# Autodesk Inventor assembly: prototype3
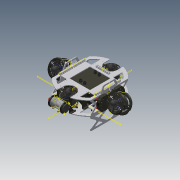
[picture p0: Inventor's stored thumbnail of the model, 180x180]
Saved by Autodesk Inventor 2018 (Build 220112000, 112)
## iProperties
Created: 2020-01-08
Part Number: prototype3
Document SubType Name: Assembly
Designer: anirudh
Author: anirudh
## Documents named in this file (33)
- D:\Silicon Sharks\2019-2020\prototype3\prototype3.iam
- D:\Silicon Sharks\2019-2020\prototype3\bottomPlate.ipt
- D:\Silicon Sharks\2019-2020\ElectronicsHousing\Prototype2\ElectricalHousing2.iam
- D:\Silicon Sharks\2019-2020\prototype3\servo.ipt
- D:\Silicon Sharks\2019-2020\prototype3\servoBracket.ipt
- D:\Silicon Sharks\2019-2020\prototype3\REV-41-1363.ipt
- D:\Silicon Sharks\2019-2020\prototype3\T200-THRUSTER.ipt
- D:\Silicon Sharks\2019-2020\prototype3\sidePlate.ipt
- D:\Silicon Sharks\2019-2020\prototype3\thrusterGimbalMount.ipt
- D:\Silicon Sharks\2019-2020\prototype3\thrusterMount.ipt
- D:\Silicon Sharks\2019-2020\prototype3\gimbalShroud.ipt
- D:\Silicon Sharks\2019-2020\prototype3\thrusterGuards.ipt
- D:\Silicon Sharks\2019-2020\prototype3\thrusterGuard2.ipt
- D:\Silicon Sharks\2019-2020\prototype3\verticalThrusterMount.ipt
- D:\Silicon Sharks\2019-2020\prototype3\topPlate.ipt
- D:\Silicon Sharks\2019-2020\CameraEnclosure\CameraEnclosure1.iam
- D:\Silicon Sharks\2019-2020\prototype3\cameraMount1.ipt
- D:\Silicon Sharks\2019-2020\prototype3\cameraMount2.ipt
- D:\Silicon Sharks\2019-2020\prototype3\cameraMount3.ipt
- D:\Silicon Sharks\2019-2020\prototype3\7inREV.ipt
- D:\Silicon Sharks\2019-2020\prototype3\4inREV.ipt
- D:\Silicon Sharks\2019-2020\prototype3\standoff.ipt
- D:\Silicon Sharks\2019-2020\prototype3\bottomMountingPlate.ipt
- D:\Silicon Sharks\2019-2020\prototype3\landingGear.ipt
- D:\Silicon Sharks\2019-2020\prototype3\bottomCameraMount.ipt
- D:\Silicon Sharks\2019-2020\prototype3\bottomCameraMount2.ipt
- D:\Silicon Sharks\2019-2020\prototype3\gimbalThrusterFrontCover.ipt
- D:\Silicon Sharks\2019-2020\prototype3\gimbalThrusterBackCover.ipt
- D:\Silicon Sharks\2019-2020\prototype3\landingGearBracket.ipt
- D:\Silicon Sharks\2019-2020\prototype3\verticalThrusterCover.ipt
- D:\Silicon Sharks\2019-2020\prototype3\verticalThrusterCover2.ipt
- D:\Silicon Sharks\2019-2020\prototype3\handle.ipt
- D:\Silicon Sharks\2019-2020\CameraEnclosure\usbCamera.ipt
## Components (68 placed, 32 different names)
1. bottomPlate:1 — Mate:1, Mate:2, Mate:3, Mate:4, Mate:5, Mate:6, Flush:1, Flush:2, Mate:13, Mate:14, Mate:15, Mate:44, Mate:45, Mate:46, Mate:50, Mate:51, Mate:52, Mate:77, Mate:78, Mate:84, Mate:85, Mate:93, Mate:96, Mate:115, Mate:116, Mate:119, Mate:120, Mate:121, Mate:122, Mate:123, Mate:124, Mate:125, Mate:126, Mate:131, Mate:132, Mate:133, Mate:134, Mate:135, Mate:136, Mate:167, Mate:168, Mate:170, Mate:171, Mate:173, Mate:174, Mate:176, Mate:177, Mate:184, Mate:185, Mate:186, Mate:187, Mate:188, Mate:189
2. ElectricalHousing2:1 [sub-assembly] — Mate:1, Mate:2, Mate:3, Mate:4, Mate:5, Mate:79, Mate:86
3. servo:1 — Mate:6, Flush:1, Flush:2, Mate:7, Mate:8, Mate:9, Mate:10, Mate:11, Mate:12, Mate:18
4. servoBracket:1 — Mate:7, Mate:8, Mate:9
5. REV-41-1363:1 — Mate:10, Mate:11, Mate:12, Mate:16, Mate:17
6. T200-THRUSTER:1 — Mate:23, Mate:24, Mate:38
7. sidePlate:1 — Mate:13, Mate:14, Mate:15, Mate:27, Mate:30, Flush:3, Mate:31, Mate:32, Flush:4, Mate:90, Mate:92
8. thrusterGimbalMount:1 — Mate:16, Mate:17, Mate:18, Mate:20, Mate:21, Mate:26, Mate:54, Mate:64
9. thrusterMount:1 — Mate:20, Mate:21, Mate:23, Mate:24, Mate:26, Mate:33, Mate:34, Mate:35, Mate:36, Mate:37
10. gimbalShroud:1 — Mate:27, Mate:30, Flush:3
11. gimbalShroud:2 — Mate:31, Mate:32, Flush:4
12. thrusterGuards:1 — Mate:33, Mate:34, Mate:35, Mate:36, Mate:37, Mate:38, Mate:39, Flush:5, Mate:40, Mate:152, Mate:154
13. thrusterGuard2:1 — Mate:39, Flush:5, Mate:40, Flush:18, Flush:19, Mate:153, Mate:155
14. servo:2 — Mate:41, Mate:42, Mate:43, Mate:47, Mate:48, Mate:49
15. servoBracket:2 — Mate:41, Mate:42, Mate:43, Mate:44, Mate:45, Mate:46
16. REV-41-1363:2 — Mate:47, Mate:48, Mate:49, Mate:53
17. sidePlate:2 — Mate:50, Mate:51, Mate:52, Mate:59, Mate:60, Flush:6, Mate:61, Mate:62, Flush:7, Mate:91, Mate:112
18. thrusterGimbalMount:2 — Mate:53, Mate:54, Mate:56, Mate:57, Mate:58, Mate:64
19. thrusterMount:2 — Mate:56, Mate:57, Mate:58, Mate:63, Mate:65, Mate:66, Mate:67, Mate:68
20. gimbalShroud:3 — Mate:61, Mate:62, Flush:7
21. gimbalShroud:4 — Mate:59, Mate:60, Flush:6
22. thrusterGuards:2 — Mate:63, Mate:65, Mate:66, Mate:67, Mate:68, Mate:70, Mate:71, Mate:72, Mate:73, Mate:74, Mate:75, Flush:8, Mate:76
23. T200-THRUSTER:2 — Mate:70, Mate:71, Mate:72, Mate:73, Mate:74
24. thrusterGuard2:2 — Mate:75, Flush:8, Mate:76, Mate:159, Mate:160, Mate:161, Mate:162
25. verticalThrusterMount:1 — Mate:77, Mate:78, Mate:79, Mate:81, Mate:82, Mate:83
26. T200-THRUSTER:3 — Mate:81, Mate:82, Mate:83
27. verticalThrusterMount:2 — Mate:84, Mate:85, Mate:86, Mate:87, Mate:88, Mate:89, Mate:114
28. T200-THRUSTER:4 — Mate:87, Mate:88, Mate:89
29. topPlate:1 — Mate:90, Mate:91, Mate:92, Mate:94, Mate:95, Mate:97, Mate:98, Mate:109, Mate:110, Mate:111, Flush:13, Flush:14, Mate:113, Flush:15, Mate:178, Mate:179, Mate:180, Mate:181, Mate:182, Mate:183, Mate:190, Mate:193
30. CameraEnclosure1:2 [sub-assembly] — Mate:103, Mate:104, Mate:197
31. cameraMount1:1 — Mate:93, Mate:94, Mate:95, Mate:101, Mate:102, Flush:10
32. cameraMount1:2 — Mate:96, Mate:97, Mate:98, Mate:99, Mate:100, Flush:9
33. cameraMount2:1 — Mate:99, Mate:100, Flush:9, Mate:106, Mate:107, Flush:12
34. cameraMount2:2 — Mate:101, Mate:102, Flush:10, Mate:103, Mate:104, Mate:105, Mate:108, Flush:11
35. cameraMount3:1 — Mate:105, Mate:108, Flush:11
36. cameraMount3:2 — Mate:106, Mate:107, Flush:12
37. 7inREV:1 — Mate:111, Mate:112, Flush:13, Mate:194, Mate:195
38. 7inREV:2 — Mate:109, Mate:110, Flush:14, Mate:191, Mate:192
39. 4inREV:1 — Mate:113, Mate:114, Flush:15
40. standoff:1 — Mate:115, Mate:116, Mate:130, Mate:139
41. standoff:2 — Mate:123, Mate:124
42. standoff:3 — Mate:121, Mate:122
43. standoff:4 — Mate:125, Mate:126
44. standoff:6 — Mate:119, Mate:120, Mate:128
45. bottomMountingPlate:1 — Mate:128, Mate:130, Mate:139, Mate:140, Mate:141, Mate:142, Mate:143, Mate:144, Mate:145
46. landingGear:1 — Mate:131, Mate:132, Mate:133, Mate:166, Mate:169
47. landingGear:2 — Mate:134, Mate:135, Mate:136, Mate:172, Mate:175
48. bottomCameraMount:1 — Mate:143, Mate:144, Mate:145, Mate:147, Mate:150, Mate:151, Flush:17
49. bottomCameraMount:2 — Mate:140, Mate:141, Mate:142, Mate:146, Mate:148, Mate:149, Flush:16
50. CameraEnclosure1:3 [sub-assembly] — Mate:146, Mate:147
51. bottomCameraMount2:1 — Mate:150, Mate:151, Flush:17
52. bottomCameraMount2:2 — Mate:148, Mate:149, Flush:16
53. gimbalThrusterFrontCover:1 — Mate:152, Mate:153
54. gimbalThrusterBackCover:1 — Mate:154, Mate:155
55. gimbalThrusterBackCover:2 — Mate:161, Mate:162, Mate:163, Mate:164, Mate:165
56. gimbalThrusterFrontCover:2 — Mate:159, Mate:160, Mate:163, Mate:164, Mate:165
57. landingGearBracket:1 — Mate:166, Mate:167, Mate:168
58. landingGearBracket:2 — Mate:172, Mate:173, Mate:174
59. landingGearBracket:3 — Mate:175, Mate:176, Mate:177
60. landingGearBracket:4 — Mate:169, Mate:170, Mate:171
61. verticalThrusterCover:1 — Mate:178, Mate:179, Mate:180
62. verticalThrusterCover:2 — Mate:181, Mate:182, Mate:183
63. verticalThrusterCover2:1 — Mate:184, Mate:185, Mate:186
64. verticalThrusterCover2:2 — Mate:187, Mate:188, Mate:189
65. handle:1 — Mate:193, Mate:194, Mate:195
66. handle:2 — Mate:190, Mate:191, Mate:192
67. cameraMount2:3 — Mate:196, Flush:20, Flush:21, Mate:197
68. usbCamera:1 — Mate:196, Flush:20, Flush:21
## Relationships (201: Mate 180, Flush 21)
- Mate:1: bottomPlate:1 ↔ ElectricalHousing2:1
- Mate:2: bottomPlate:1 ↔ ElectricalHousing2:1
- Mate:3: bottomPlate:1 ↔ ElectricalHousing2:1
- Mate:4: bottomPlate:1 ↔ ElectricalHousing2:1
- Mate:5: bottomPlate:1 ↔ ElectricalHousing2:1
- Mate:6: bottomPlate:1 ↔ servo:1
- Flush:1 (-50.8 mm): bottomPlate:1 ↔ servo:1
- Flush:2: bottomPlate:1 ↔ servo:1
- Mate:7: servo:1 ↔ servoBracket:1
- Mate:8 (0.65 mm): servo:1 ↔ servoBracket:1
- Mate:9 (0.7 mm): servo:1 ↔ servoBracket:1
- Mate:10: servo:1 ↔ REV-41-1363:1
- Mate:11: servo:1 ↔ REV-41-1363:1
- Mate:12: servo:1 ↔ REV-41-1363:1
- Mate:13: bottomPlate:1 ↔ sidePlate:1
- Mate:14: bottomPlate:1 ↔ sidePlate:1
- Mate:15: bottomPlate:1 ↔ sidePlate:1
- Mate:16: REV-41-1363:1 ↔ thrusterGimbalMount:1
- Mate:17: REV-41-1363:1 ↔ thrusterGimbalMount:1
- Mate:18: servo:1 ↔ thrusterGimbalMount:1
- Mate:20: thrusterGimbalMount:1 ↔ thrusterMount:1
- Mate:21: thrusterGimbalMount:1 ↔ thrusterMount:1
- Mate:23: T200-THRUSTER:1 ↔ thrusterMount:1
- Mate:24: T200-THRUSTER:1 ↔ thrusterMount:1
- Mate:26: thrusterGimbalMount:1 ↔ thrusterMount:1
- Mate:27: sidePlate:1 ↔ gimbalShroud:1
- Mate:30: sidePlate:1 ↔ gimbalShroud:1
- Flush:3: sidePlate:1 ↔ gimbalShroud:1
- Mate:31: sidePlate:1 ↔ gimbalShroud:2
- Mate:32: sidePlate:1 ↔ gimbalShroud:2
- Flush:4: sidePlate:1 ↔ gimbalShroud:2
- Mate:33: thrusterMount:1 ↔ thrusterGuards:1
- Mate:34: thrusterMount:1 ↔ thrusterGuards:1
- Mate:35: thrusterMount:1 ↔ thrusterGuards:1
- Mate:36: thrusterMount:1 ↔ thrusterGuards:1
- Mate:37: thrusterMount:1 ↔ thrusterGuards:1
- Mate:38: T200-THRUSTER:1 ↔ thrusterGuards:1
- Mate:39: thrusterGuards:1 ↔ thrusterGuard2:1
- Flush:5: thrusterGuards:1 ↔ thrusterGuard2:1
- Mate:40: thrusterGuards:1 ↔ thrusterGuard2:1
- Mate:41: servo:2 ↔ servoBracket:2
- Mate:42 (0.7112 mm): servo:2 ↔ servoBracket:2
- Mate:43 (0.6477 mm): servo:2 ↔ servoBracket:2
- Mate:44: bottomPlate:1 ↔ servoBracket:2
- Mate:45: bottomPlate:1 ↔ servoBracket:2
- Mate:46: bottomPlate:1 ↔ servoBracket:2
- Mate:47: servo:2 ↔ REV-41-1363:2
- Mate:48: servo:2 ↔ REV-41-1363:2
- Mate:49: servo:2 ↔ REV-41-1363:2
- Mate:50: bottomPlate:1 ↔ sidePlate:2
- Mate:51: bottomPlate:1 ↔ sidePlate:2
- Mate:52: bottomPlate:1 ↔ sidePlate:2
- Mate:53: REV-41-1363:2 ↔ thrusterGimbalMount:2
- Mate:54: thrusterGimbalMount:1 ↔ thrusterGimbalMount:2
- Mate:56: thrusterGimbalMount:2 ↔ thrusterMount:2
- Mate:57: thrusterGimbalMount:2 ↔ thrusterMount:2
- Mate:58: thrusterGimbalMount:2 ↔ thrusterMount:2
- Mate:59: sidePlate:2 ↔ gimbalShroud:4
- Mate:60: sidePlate:2 ↔ gimbalShroud:4
- Flush:6: sidePlate:2 ↔ gimbalShroud:4
- Mate:61: sidePlate:2 ↔ gimbalShroud:3
- Mate:62: sidePlate:2 ↔ gimbalShroud:3
- Flush:7: sidePlate:2 ↔ gimbalShroud:3
- Mate:63: thrusterMount:2 ↔ thrusterGuards:2
- Mate:64: thrusterGimbalMount:1 ↔ thrusterGimbalMount:2
- Mate:65: thrusterMount:2 ↔ thrusterGuards:2
- Mate:66: thrusterMount:2 ↔ thrusterGuards:2
- Mate:67: thrusterMount:2 ↔ thrusterGuards:2
- Mate:68: thrusterMount:2 ↔ thrusterGuards:2
- Mate:70: thrusterGuards:2 ↔ T200-THRUSTER:2
- Mate:71: thrusterGuards:2 ↔ T200-THRUSTER:2
- Mate:72: thrusterGuards:2 ↔ T200-THRUSTER:2
- Mate:73: thrusterGuards:2 ↔ T200-THRUSTER:2
- Mate:74: thrusterGuards:2 ↔ T200-THRUSTER:2
- Mate:75: thrusterGuards:2 ↔ thrusterGuard2:2
- Flush:8: thrusterGuards:2 ↔ thrusterGuard2:2
- Mate:76: thrusterGuards:2 ↔ thrusterGuard2:2
- Mate:77: bottomPlate:1 ↔ verticalThrusterMount:1
- Mate:78: bottomPlate:1 ↔ verticalThrusterMount:1
- Mate:79 (3.175 mm): ElectricalHousing2:1 ↔ verticalThrusterMount:1
- Mate:81: verticalThrusterMount:1 ↔ T200-THRUSTER:3
- Mate:82: verticalThrusterMount:1 ↔ T200-THRUSTER:3
- Mate:83: verticalThrusterMount:1 ↔ T200-THRUSTER:3
- Mate:84: bottomPlate:1 ↔ verticalThrusterMount:2
- Mate:85: bottomPlate:1 ↔ verticalThrusterMount:2
- Mate:86 (3.175 mm): ElectricalHousing2:1 ↔ verticalThrusterMount:2
- Mate:87: verticalThrusterMount:2 ↔ T200-THRUSTER:4
- Mate:88: verticalThrusterMount:2 ↔ T200-THRUSTER:4
- Mate:89: verticalThrusterMount:2 ↔ T200-THRUSTER:4
- Mate:90: sidePlate:1 ↔ topPlate:1
- Mate:91: sidePlate:2 ↔ topPlate:1
- Mate:92: sidePlate:1 ↔ topPlate:1
- Mate:93: bottomPlate:1 ↔ cameraMount1:1
- Mate:94: topPlate:1 ↔ cameraMount1:1
- Mate:95: topPlate:1 ↔ cameraMount1:1
- Mate:96: bottomPlate:1 ↔ cameraMount1:2
- Mate:97: topPlate:1 ↔ cameraMount1:2
- Mate:98: topPlate:1 ↔ cameraMount1:2
- Mate:99: cameraMount1:2 ↔ cameraMount2:1
- Mate:100: cameraMount1:2 ↔ cameraMount2:1
- Mate:101: cameraMount1:1 ↔ cameraMount2:2
- Mate:102: cameraMount1:1 ↔ cameraMount2:2
- Flush:9: cameraMount1:2 ↔ cameraMount2:1
- Flush:10: cameraMount1:1 ↔ cameraMount2:2
- Mate:103 (-0.0381 mm): CameraEnclosure1:2 ↔ cameraMount2:2
- Mate:104: CameraEnclosure1:2 ↔ cameraMount2:2
- Mate:105: cameraMount2:2 ↔ cameraMount3:1
- Mate:106: cameraMount2:1 ↔ cameraMount3:2
- Mate:107: cameraMount2:1 ↔ cameraMount3:2
- Mate:108: cameraMount2:2 ↔ cameraMount3:1
- Flush:11: cameraMount2:2 ↔ cameraMount3:1
- Flush:12: cameraMount2:1 ↔ cameraMount3:2
- Mate:109: topPlate:1 ↔ 7inREV:2
- Mate:110: topPlate:1 ↔ 7inREV:2
- Mate:111: topPlate:1 ↔ 7inREV:1
- Mate:112: sidePlate:2 ↔ 7inREV:1
- Flush:13 (-0.8128 mm): topPlate:1 ↔ 7inREV:1
- Flush:14 (-0.8128 mm): topPlate:1 ↔ 7inREV:2
- Mate:113: topPlate:1 ↔ 4inREV:1
- Mate:114: verticalThrusterMount:2 ↔ 4inREV:1
- Flush:15 (15 mm): topPlate:1 ↔ 4inREV:1
- Mate:115: bottomPlate:1 ↔ standoff:1
- Mate:116: bottomPlate:1 ↔ standoff:1
- Mate:119: bottomPlate:1 ↔ standoff:6
- Mate:120: bottomPlate:1 ↔ standoff:6
- Mate:121: bottomPlate:1 ↔ standoff:3
- Mate:122: bottomPlate:1 ↔ standoff:3
- Mate:123: bottomPlate:1 ↔ standoff:2
- Mate:124: bottomPlate:1 ↔ standoff:2
- Mate:125: bottomPlate:1 ↔ standoff:4
- Mate:126: bottomPlate:1 ↔ standoff:4
- Mate:128: standoff:6 ↔ bottomMountingPlate:1
- Mate:130: standoff:1 ↔ bottomMountingPlate:1
- Mate:131: bottomPlate:1 ↔ landingGear:1
- Mate:132: bottomPlate:1 ↔ landingGear:1
- Mate:133: bottomPlate:1 ↔ landingGear:1
- Mate:134: bottomPlate:1 ↔ landingGear:2
- Mate:135: bottomPlate:1 ↔ landingGear:2
- Mate:136: bottomPlate:1 ↔ landingGear:2
- Mate:139: standoff:1 ↔ bottomMountingPlate:1
- Mate:140: bottomMountingPlate:1 ↔ bottomCameraMount:2
- Mate:141: bottomMountingPlate:1 ↔ bottomCameraMount:2
- Mate:142: bottomMountingPlate:1 ↔ bottomCameraMount:2
- Mate:143: bottomMountingPlate:1 ↔ bottomCameraMount:1
- Mate:144: bottomMountingPlate:1 ↔ bottomCameraMount:1
- Mate:145: bottomMountingPlate:1 ↔ bottomCameraMount:1
- Mate:146: bottomCameraMount:2 ↔ CameraEnclosure1:3
- Mate:147: bottomCameraMount:1 ↔ CameraEnclosure1:3
- Mate:148: bottomCameraMount:2 ↔ bottomCameraMount2:2
- Mate:149: bottomCameraMount:2 ↔ bottomCameraMount2:2
- Flush:16: bottomCameraMount:2 ↔ bottomCameraMount2:2
- Mate:150: bottomCameraMount:1 ↔ bottomCameraMount2:1
- Mate:151: bottomCameraMount:1 ↔ bottomCameraMount2:1
- Flush:17: bottomCameraMount:1 ↔ bottomCameraMount2:1
- Flush:18 (5.08 mm): thrusterGuard2:1
- Flush:19 (5.08 mm): thrusterGuard2:1
- Mate:152: thrusterGuards:1 ↔ gimbalThrusterFrontCover:1
- Mate:153: thrusterGuard2:1 ↔ gimbalThrusterFrontCover:1
- Mate:154: thrusterGuards:1 ↔ gimbalThrusterBackCover:1
- Mate:155: thrusterGuard2:1 ↔ gimbalThrusterBackCover:1
- Mate:159: thrusterGuard2:2 ↔ gimbalThrusterFrontCover:2
- Mate:160: thrusterGuard2:2 ↔ gimbalThrusterFrontCover:2
- Mate:161: thrusterGuard2:2 ↔ gimbalThrusterBackCover:2
- Mate:162: thrusterGuard2:2 ↔ gimbalThrusterBackCover:2
- Mate:163: gimbalThrusterBackCover:2 ↔ gimbalThrusterFrontCover:2
- Mate:164: gimbalThrusterBackCover:2 ↔ gimbalThrusterFrontCover:2
- Mate:165: gimbalThrusterBackCover:2 ↔ gimbalThrusterFrontCover:2
- Mate:166: landingGear:1 ↔ landingGearBracket:1
- Mate:167: bottomPlate:1 ↔ landingGearBracket:1
- Mate:168: bottomPlate:1 ↔ landingGearBracket:1
- Mate:169: landingGear:1 ↔ landingGearBracket:4
- Mate:170: bottomPlate:1 ↔ landingGearBracket:4
- Mate:171: bottomPlate:1 ↔ landingGearBracket:4
- Mate:172: landingGear:2 ↔ landingGearBracket:2
- Mate:173: bottomPlate:1 ↔ landingGearBracket:2
- Mate:174: bottomPlate:1 ↔ landingGearBracket:2
- Mate:175: landingGear:2 ↔ landingGearBracket:3
- Mate:176: bottomPlate:1 ↔ landingGearBracket:3
- Mate:177: bottomPlate:1 ↔ landingGearBracket:3
- Mate:178 (11.43 mm): topPlate:1 ↔ verticalThrusterCover:1
- Mate:179: topPlate:1 ↔ verticalThrusterCover:1
- Mate:180: topPlate:1 ↔ verticalThrusterCover:1
- Mate:181 (11.43 mm): topPlate:1 ↔ verticalThrusterCover:2
- Mate:182: topPlate:1 ↔ verticalThrusterCover:2
- Mate:183: topPlate:1 ↔ verticalThrusterCover:2
- Mate:184 (20 mm): bottomPlate:1 ↔ verticalThrusterCover2:1
- Mate:185: bottomPlate:1 ↔ verticalThrusterCover2:1
- Mate:186: bottomPlate:1 ↔ verticalThrusterCover2:1
- Mate:187 (20 mm): bottomPlate:1 ↔ verticalThrusterCover2:2
- Mate:188: bottomPlate:1 ↔ verticalThrusterCover2:2
- Mate:189: bottomPlate:1 ↔ verticalThrusterCover2:2
- Mate:190: topPlate:1 ↔ handle:2
- Mate:191: 7inREV:2 ↔ handle:2
- Mate:192: 7inREV:2 ↔ handle:2
- Mate:193: topPlate:1 ↔ handle:1
- Mate:194: 7inREV:1 ↔ handle:1
- Mate:195: 7inREV:1 ↔ handle:1
- Mate:196: cameraMount2:3 ↔ usbCamera:1
- Flush:20 (2.2606 mm): cameraMount2:3 ↔ usbCamera:1
- Flush:21 (2.0574 mm): cameraMount2:3 ↔ usbCamera:1
- Mate:197: CameraEnclosure1:2 ↔ cameraMount2:3
